# Autodesk Inventor assembly: Assembly1
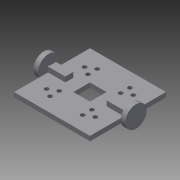
[picture p0: Inventor's stored thumbnail of the model, 180x180]
Saved by Autodesk Inventor 2015 (Build 190159000, 159)
## iProperties
Created: 2015-04-05
Part Number: Assembly1
Document SubType Name: Assembly
Designer: Jesse
Author: Jesse
## Documents named in this file (4)
- C:\Users\Jesse\Programs\Tortuga\3D_Models\Assembly1.iam
- C:\Users\Jesse\Programs\Tortuga\3D_Models\Prototype1.ipt
- C:\Users\Jesse\Programs\Tortuga\3D_Models\Motor.ipt
- C:\Users\Jesse\Programs\Tortuga\3D_Models\BallCaster.ipt
## Components (5 placed, 3 different names)
1. Prototype1:1 — Mate:1, Mate:2, Mate:3, Mate:4, Mate:5, Mate:6, Mate:7, Mate:8
2. Motor:1 — Mate:3, Mate:4, Mate:5
3. Motor:3 — Mate:1, Mate:2, Mate:6
4. BallCaster:1 — Mate:7
5. BallCaster:2 — Mate:8
## Relationships (8: Mate 8)
- Mate:1: Prototype1:1 ↔ Motor:3
- Mate:2: Prototype1:1 ↔ Motor:3
- Mate:3: Prototype1:1 ↔ Motor:1
- Mate:4: Prototype1:1 ↔ Motor:1
- Mate:5: Prototype1:1 ↔ Motor:1
- Mate:6: Prototype1:1 ↔ Motor:3
- Mate:7: Prototype1:1 ↔ BallCaster:1
- Mate:8: Prototype1:1 ↔ BallCaster:2
